# Autodesk Inventor assembly: noga_pre
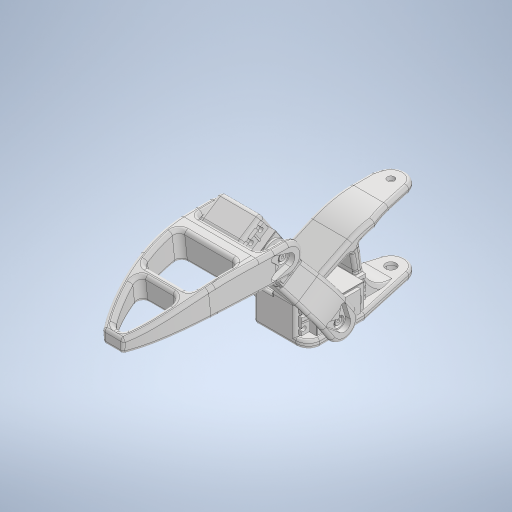
[picture p0: Inventor's stored thumbnail of the model, 512x512]
Saved by Autodesk Inventor 2023 (Build 270158000, 158)
## iProperties
Created: 2024-06-27
Part Number: noga_pre
Document SubType Name: Assembly
Designer: kamil
Author: kamil
## Documents named in this file (9)
- C:\Users\kamil\Documents\PROJECTS - repos\Robal-2.0\mechanics\noga_pre.iam
- C:\Users\kamil\Documents\PROJECTS - repos\Robal-2.0\mechanics\Standard-Servo.ipt
- C:\Users\kamil\Documents\PROJECTS - repos\Robal-2.0\mechanics\blacha_dolna_pre.ipt
- C:\Users\kamil\Documents\PROJECTS - repos\Robal-2.0\mechanics\blacha_gorna_pre.ipt
- C:\Users\kamil\Documents\PROJECTS - repos\Robal-2.0\mechanics\uchwyt_serwa_czlon1_pre.ipt
- C:\Users\kamil\Documents\PROJECTS - repos\Robal-2.0\mechanics\czlon2_pre.ipt
- C:\Users\kamil\Documents\PROJECTS - repos\Robal-2.0\mechanics\czlon3_pre.ipt
- C:\Users\kamil\Documents\PROJECTS - repos\Robal-2.0\mechanics\czlon4_pre.ipt
- C:\Users\kamil\Documents\PROJECTS - repos\Robal-2.0\mechanics\czlon4_pre_2.ipt
## Components (10 placed, 8 different names)
1. Standard-Servo:1 — Zestawiające:9, Zestawiające:10, Zestawiające:11, Zestawiające:12
2. Standard-Servo:2 — Zestawiające:1, Równoległe:1, Zestawiające:2, Zestawiające:7, Zestawiające:8
3. blacha_dolna_pre:1 — Zestawiające:3, Równoległe:2, Zestawiające:4
4. blacha_gorna_pre:1 — Zestawiające:5, Równoległe:3, Zestawiające:6
5. uchwyt_serwa_czlon1_pre:1 — Zestawiające:1, Równoległe:1, Zestawiające:2, Zestawiające:3, Równoległe:2, Zestawiające:4, Zestawiające:5, Równoległe:3, Zestawiające:6
6. czlon2_pre:1 — Zestawiające:7, Zestawiające:8, Zestawiające:9, Zestawiające:10, Zestawiające:11, Zestawiające:13
7. czlon3_pre:1 — Zestawiające:12, Zestawiające:13, Zestawiające:17, Zestawiające:21, Równoległe:4
8. Standard-Servo:3 — Zestawiające:17, Zestawiające:21, Równoległe:4, Zestawiające:22, Zestawiające:23
9. czlon4_pre:1
10. czlon4_pre_2:1 — Zestawiające:22, Zestawiające:23
## Relationships (21: Mate 17, Flush 4)
- Zestawiające:1 [Mate]: Standard-Servo:2 ↔ uchwyt_serwa_czlon1_pre:1
- Równoległe:1 [Flush]: Standard-Servo:2 ↔ uchwyt_serwa_czlon1_pre:1
- Zestawiające:2 [Mate] (1 mm): Standard-Servo:2 ↔ uchwyt_serwa_czlon1_pre:1
- Zestawiające:3 [Mate]: blacha_dolna_pre:1 ↔ uchwyt_serwa_czlon1_pre:1
- Równoległe:2 [Flush]: blacha_dolna_pre:1 ↔ uchwyt_serwa_czlon1_pre:1
- Zestawiające:4 [Mate]: blacha_dolna_pre:1 ↔ uchwyt_serwa_czlon1_pre:1
- Zestawiające:5 [Mate]: blacha_gorna_pre:1 ↔ uchwyt_serwa_czlon1_pre:1
- Równoległe:3 [Flush]: blacha_gorna_pre:1 ↔ uchwyt_serwa_czlon1_pre:1
- Zestawiające:6 [Mate]: blacha_gorna_pre:1 ↔ uchwyt_serwa_czlon1_pre:1
- Zestawiające:7 [Mate] (2.1 mm): Standard-Servo:2 ↔ czlon2_pre:1
- Zestawiające:8 [Mate]: Standard-Servo:2 ↔ czlon2_pre:1
- Zestawiające:9 [Mate] (1 mm): Standard-Servo:1 ↔ czlon2_pre:1
- Zestawiające:10 [Mate] (1 mm): Standard-Servo:1 ↔ czlon2_pre:1
- Zestawiające:11 [Mate]: Standard-Servo:1 ↔ czlon2_pre:1
- Zestawiające:12 [Mate] (2.1 mm): Standard-Servo:1 ↔ czlon3_pre:1
- Zestawiające:13 [Mate]: czlon2_pre:1 ↔ czlon3_pre:1
- Zestawiające:17 [Mate] (1 mm): czlon3_pre:1 ↔ Standard-Servo:3
- Zestawiające:21 [Mate]: czlon3_pre:1 ↔ Standard-Servo:3
- Równoległe:4 [Flush]: czlon3_pre:1 ↔ Standard-Servo:3
- Zestawiające:22 [Mate] (2.1 mm): Standard-Servo:3 ↔ czlon4_pre_2:1
- Zestawiające:23 [Mate]: Standard-Servo:3 ↔ czlon4_pre_2:1
